# Autodesk Inventor assembly: termoformadora
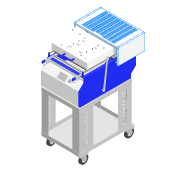
[picture p0: Inventor's stored thumbnail of the model, 180x180]
Saved by Autodesk Inventor 2021 (Build 250183000, 183)
## iProperties
Created: 2021-04-15
Part Number: termoformadora
Document SubType Name: Assembly
Designer: Leonardo Fabio Mercado Benítez
Author: Leonardo Fabio Mercado Benítez
## Documents named in this file (18)
- E:\Documentos\Documentos\Michael_Rodriguez\Universidad_Nacional\Doceaba matricula\PAI\Proyecto PAI\Proyecto_PAI_2021\01 CAD\termoformadora.iam
- E:\Documentos\Documentos\Michael_Rodriguez\Universidad_Nacional\Doceaba matricula\PAI\Proyecto PAI\Proyecto_PAI_2021\01 CAD\Ensamblaje carcasa superior.iam
- E:\Documentos\Documentos\Michael_Rodriguez\Universidad_Nacional\Doceaba matricula\PAI\Proyecto PAI\Proyecto_PAI_2021\01 CAD\soporte_inferior_zona_calor.ipt
- E:\Documentos\Documentos\Michael_Rodriguez\Universidad_Nacional\Doceaba matricula\PAI\Proyecto PAI\Proyecto_PAI_2021\01 CAD\tapa_caja_calor.ipt
- E:\Documentos\Documentos\Michael_Rodriguez\Universidad_Nacional\Doceaba matricula\PAI\Proyecto PAI\Proyecto_PAI_2021\01 CAD\angulo_caja_calor.ipt
- E:\Documentos\Documentos\Michael_Rodriguez\Universidad_Nacional\Doceaba matricula\PAI\Proyecto PAI\Proyecto_PAI_2021\01 CAD\buje_carro_zona_calor.ipt
- E:\Documentos\Documentos\Michael_Rodriguez\Universidad_Nacional\Doceaba matricula\PAI\Proyecto PAI\Proyecto_PAI_2021\01 CAD\barra.ipt
- E:\Documentos\Documentos\Michael_Rodriguez\Universidad_Nacional\Doceaba matricula\PAI\Proyecto PAI\Proyecto_PAI_2021\01 CAD\mango_zona_calor.ipt
- E:\Documentos\Documentos\Michael_Rodriguez\Universidad_Nacional\Doceaba matricula\PAI\Proyecto PAI\Proyecto_PAI_2021\01 CAD\Ensamblaje carcasa control.iam
- E:\Documentos\Documentos\Michael_Rodriguez\Universidad_Nacional\Doceaba matricula\PAI\Proyecto PAI\Proyecto_PAI_2021\01 CAD\soporte_barra.ipt
- E:\Documentos\Documentos\Michael_Rodriguez\Universidad_Nacional\Doceaba matricula\PAI\Proyecto PAI\Proyecto_PAI_2021\01 CAD\ensamble resistencias.iam
- E:\Documentos\Documentos\Michael_Rodriguez\Universidad_Nacional\Doceaba matricula\PAI\Proyecto PAI\Proyecto_PAI_2021\01 CAD\soporte_resistencias.ipt
- E:\Documentos\Documentos\Michael_Rodriguez\Universidad_Nacional\Doceaba matricula\PAI\Proyecto PAI\Proyecto_PAI_2021\01 CAD\Estructura Lámina.iam
- E:\Documentos\Documentos\Michael_Rodriguez\Universidad_Nacional\Doceaba matricula\PAI\Proyecto PAI\Proyecto_PAI_2021\01 CAD\conector_ceramico.ipt
- E:\Documentos\Documentos\Michael_Rodriguez\Universidad_Nacional\Doceaba matricula\PAI\Proyecto PAI\Proyecto_PAI_2021\01 CAD\guarda_conector_ceramico.ipt
- E:\Documentos\Documentos\Michael_Rodriguez\Universidad_Nacional\Doceaba matricula\PAI\Proyecto PAI\Proyecto_PAI_2021\01 CAD\guarda_cables.ipt
- E:\Documentos\Documentos\Michael_Rodriguez\Universidad_Nacional\Doceaba matricula\PAI\Proyecto PAI\Proyecto_PAI_2021\01 CAD\Barras_Soporte_superior.ipt
- C:\Users\Admin\Documents\Inventor\Content Center Files\R2021\es-ES\ISO 7380-1\ISO 7380-1 - M5 x 16.ipt
## Components (34 placed, 17 different names)
1. Ensamblaje carcasa superior:1 [sub-assembly] — Coincidencia:1, Coincidencia:2, Coincidencia:11, Coincidencia:12, Nivelación:7, Coincidencia:16, Coincidencia:17, Coincidencia:57, Coincidencia:58, Coincidencia:59, Coincidencia:60
2. soporte_inferior_zona_calor:1 — Coincidencia:1, Coincidencia:2, Coincidencia:3, Coincidencia:5, Nivelación:3, Nivelación:4, Coincidencia:6, Nivelación:5, Nivelación:6, Coincidencia:15, Insertar:5, Insertar:6, Coincidencia:44, Coincidencia:45, Nivelación:14, Nivelación:15, Ángulo:6, Ángulo:7, Ángulo:8, Ángulo:9, Ángulo:10, Nivelación:16, Coincidencia:56, Nivelación:17
3. tapa_caja_calor:1 — Coincidencia:3, Nivelación:14, Nivelación:15
4. angulo_caja_calor:1 — Coincidencia:5, Nivelación:3, Nivelación:4, Coincidencia:7, Coincidencia:8, Insertar:1, Insertar:2
5. angulo_caja_calor:2 — Coincidencia:6, Nivelación:5, Nivelación:6, Coincidencia:9, Coincidencia:10, Insertar:3, Insertar:4
6. buje_carro_zona_calor:1 — Coincidencia:9, Insertar:3
7. buje_carro_zona_calor:2 — Coincidencia:8, Insertar:2, Coincidencia:14
8. buje_carro_zona_calor:3 — Coincidencia:10, Insertar:4
9. buje_carro_zona_calor:4 — Coincidencia:7, Insertar:1, Coincidencia:13
10. barra:1 — Coincidencia:11, Coincidencia:13, Coincidencia:21
11. barra:2 — Coincidencia:12, Coincidencia:14, Coincidencia:22
12. mango_zona_calor:1 — Coincidencia:15, Insertar:5, Insertar:6
13. Ensamblaje carcasa control:1 [sub-assembly] — Nivelación:7, Coincidencia:16, Coincidencia:17, Nivelación:8, Coincidencia:18, Coincidencia:20, Nivelación:9, Coincidencia:23, Coincidencia:33, Nivelación:10, Nivelación:11
14. soporte_barra:1 — Nivelación:8, Coincidencia:18, Coincidencia:22
15. soporte_barra:2 — Coincidencia:20, Nivelación:9, Coincidencia:21
16. ensamble resistencias:1 [sub-assembly] — Coincidencia:23, Coincidencia:29, Nivelación:12, Nivelación:13
17. soporte_resistencias:1 — Coincidencia:29, Nivelación:12, Nivelación:13, Coincidencia:34, Coincidencia:35, Coincidencia:36, Coincidencia:37, Coincidencia:38, Coincidencia:39, Coincidencia:40, Coincidencia:41, Coincidencia:42, Coincidencia:43, Ángulo:1, Ángulo:2, Ángulo:3, Ángulo:4, Ángulo:5, Coincidencia:44, Coincidencia:45
18. Estructura Lámina:1 [sub-assembly] — Coincidencia:33, Nivelación:10, Nivelación:11
19. conector_ceramico:1 — Coincidencia:37, Coincidencia:42, Ángulo:2, Coincidencia:52
20. conector_ceramico:2 — Coincidencia:36, Coincidencia:41, Ángulo:1, Coincidencia:53
21. conector_ceramico:3 — Coincidencia:34, Coincidencia:39, Ángulo:4, Coincidencia:55
22. conector_ceramico:4 — Coincidencia:38, Coincidencia:43, Ángulo:5, Coincidencia:46, Coincidencia:47, Coincidencia:48, Coincidencia:49, Coincidencia:50, Coincidencia:51
23. conector_ceramico:5 — Coincidencia:35, Coincidencia:40, Ángulo:3, Coincidencia:54
24. guarda_conector_ceramico:1 — Coincidencia:46, Coincidencia:51, Ángulo:10
25. guarda_conector_ceramico:2 — Coincidencia:48, Coincidencia:54, Ángulo:8
26. guarda_conector_ceramico:3 — Coincidencia:47, Coincidencia:52, Ángulo:6
27. guarda_conector_ceramico:4 — Coincidencia:50, Coincidencia:55, Ángulo:9
28. guarda_conector_ceramico:5 — Coincidencia:49, Coincidencia:53, Ángulo:7
29. guarda_cables:1 — Nivelación:16, Coincidencia:56, Nivelación:17
30. Barras_Soporte_superior:1 — Coincidencia:57
31. Barras_Soporte_superior:2 — Coincidencia:58
32. Barras_Soporte_superior:3 — Coincidencia:60
33. Barras_Soporte_superior:4 — Coincidencia:59
34. ISO 7380-1 M5 x 16:4
## Relationships (81: Mate 50, Flush 15, Angle 10, Insert 6)
- Coincidencia:1 [Mate] (61.24 mm): Ensamblaje carcasa superior:1 ↔ soporte_inferior_zona_calor:1
- Coincidencia:2 [Mate] (29 mm): Ensamblaje carcasa superior:1 ↔ soporte_inferior_zona_calor:1
- Coincidencia:3 [Mate]: soporte_inferior_zona_calor:1 ↔ tapa_caja_calor:1
- Coincidencia:5 [Mate]: soporte_inferior_zona_calor:1 ↔ angulo_caja_calor:1
- Nivelación:3 [Flush]: soporte_inferior_zona_calor:1 ↔ angulo_caja_calor:1
- Nivelación:4 [Flush] (10 mm): soporte_inferior_zona_calor:1 ↔ angulo_caja_calor:1
- Coincidencia:6 [Mate]: soporte_inferior_zona_calor:1 ↔ angulo_caja_calor:2
- Nivelación:5 [Flush]: soporte_inferior_zona_calor:1 ↔ angulo_caja_calor:2
- Nivelación:6 [Flush]: soporte_inferior_zona_calor:1 ↔ angulo_caja_calor:2
- Coincidencia:7 [Mate]: angulo_caja_calor:1 ↔ buje_carro_zona_calor:4
- Coincidencia:8 [Mate]: angulo_caja_calor:1 ↔ buje_carro_zona_calor:2
- Coincidencia:9 [Mate]: angulo_caja_calor:2 ↔ buje_carro_zona_calor:1
- Coincidencia:10 [Mate]: angulo_caja_calor:2 ↔ buje_carro_zona_calor:3
- Insertar:1: angulo_caja_calor:1 ↔ buje_carro_zona_calor:4
- Insertar:2: angulo_caja_calor:1 ↔ buje_carro_zona_calor:2
- Insertar:3: angulo_caja_calor:2 ↔ buje_carro_zona_calor:1
- Insertar:4: angulo_caja_calor:2 ↔ buje_carro_zona_calor:3
- Coincidencia:11 [Mate]: Ensamblaje carcasa superior:1 ↔ barra:1
- Coincidencia:12 [Mate]: Ensamblaje carcasa superior:1 ↔ barra:2
- Coincidencia:13 [Mate]: buje_carro_zona_calor:4 ↔ barra:1
- Coincidencia:14 [Mate]: buje_carro_zona_calor:2 ↔ barra:2
- Coincidencia:15 [Mate]: soporte_inferior_zona_calor:1 ↔ mango_zona_calor:1
- Insertar:5: soporte_inferior_zona_calor:1 ↔ mango_zona_calor:1
- Insertar:6: soporte_inferior_zona_calor:1 ↔ mango_zona_calor:1
- Nivelación:7 [Flush] (-74.1 mm): Ensamblaje carcasa superior:1 ↔ Ensamblaje carcasa control:1
- Coincidencia:16 [Mate] (-43.5 mm): Ensamblaje carcasa superior:1 ↔ Ensamblaje carcasa control:1
- Coincidencia:17 [Mate] (53.74 mm): Ensamblaje carcasa superior:1 ↔ Ensamblaje carcasa control:1
- Nivelación:8 [Flush] (5 mm): Ensamblaje carcasa control:1 ↔ soporte_barra:1
- Coincidencia:18 [Mate]: Ensamblaje carcasa control:1 ↔ soporte_barra:1
- Coincidencia:20 [Mate]: Ensamblaje carcasa control:1 ↔ soporte_barra:2
- Nivelación:9 [Flush] (5 mm): Ensamblaje carcasa control:1 ↔ soporte_barra:2
- Coincidencia:21 [Mate]: barra:1 ↔ soporte_barra:2
- Coincidencia:22 [Mate]: barra:2 ↔ soporte_barra:1
- Coincidencia:23 [Mate] (106 mm): Ensamblaje carcasa control:1 ↔ ensamble resistencias:1
- Coincidencia:29 [Mate]: ensamble resistencias:1 ↔ soporte_resistencias:1
- Coincidencia:33 [Mate]: Ensamblaje carcasa control:1 ↔ Estructura Lámina:1
- Nivelación:10 [Flush] (10 mm): Ensamblaje carcasa control:1 ↔ Estructura Lámina:1
- Nivelación:11 [Flush]: Ensamblaje carcasa control:1 ↔ Estructura Lámina:1
- Nivelación:12 [Flush] (33.5 mm): ensamble resistencias:1 ↔ soporte_resistencias:1
- Nivelación:13 [Flush] (34 mm): ensamble resistencias:1 ↔ soporte_resistencias:1
- Coincidencia:34 [Mate]: soporte_resistencias:1 ↔ conector_ceramico:3
- Coincidencia:35 [Mate]: soporte_resistencias:1 ↔ conector_ceramico:5
- Coincidencia:36 [Mate]: soporte_resistencias:1 ↔ conector_ceramico:2
- Coincidencia:37 [Mate]: soporte_resistencias:1 ↔ conector_ceramico:1
- Coincidencia:38 [Mate]: soporte_resistencias:1 ↔ conector_ceramico:4
- Coincidencia:39 [Mate]: soporte_resistencias:1 ↔ conector_ceramico:3
- Coincidencia:40 [Mate]: soporte_resistencias:1 ↔ conector_ceramico:5
- Coincidencia:41 [Mate]: soporte_resistencias:1 ↔ conector_ceramico:2
- Coincidencia:42 [Mate]: soporte_resistencias:1 ↔ conector_ceramico:1
- Coincidencia:43 [Mate]: soporte_resistencias:1 ↔ conector_ceramico:4
- Ángulo:1 [Angle] (0 deg): soporte_resistencias:1 ↔ conector_ceramico:2
- Ángulo:2 [Angle] (0 deg): soporte_resistencias:1 ↔ conector_ceramico:1
- Ángulo:3 [Angle] (0 deg): soporte_resistencias:1 ↔ conector_ceramico:5
- Ángulo:4 [Angle] (0 deg): soporte_resistencias:1 ↔ conector_ceramico:3
- Ángulo:5 [Angle] (0 deg): soporte_resistencias:1 ↔ conector_ceramico:4
- Coincidencia:44 [Mate] (0.5 mm): soporte_inferior_zona_calor:1 ↔ soporte_resistencias:1
- Coincidencia:45 [Mate] (0.5 mm): soporte_inferior_zona_calor:1 ↔ soporte_resistencias:1
- Nivelación:14 [Flush] (25.4 mm): soporte_inferior_zona_calor:1 ↔ tapa_caja_calor:1
- Nivelación:15 [Flush] (31.75 mm): soporte_inferior_zona_calor:1 ↔ tapa_caja_calor:1
- Coincidencia:46 [Mate]: conector_ceramico:4 ↔ guarda_conector_ceramico:1
- Coincidencia:47 [Mate]: conector_ceramico:4 ↔ guarda_conector_ceramico:3
- Coincidencia:48 [Mate]: conector_ceramico:4 ↔ guarda_conector_ceramico:2
- Coincidencia:49 [Mate]: conector_ceramico:4 ↔ guarda_conector_ceramico:5
- Coincidencia:50 [Mate]: conector_ceramico:4 ↔ guarda_conector_ceramico:4
- Coincidencia:51 [Mate]: conector_ceramico:4 ↔ guarda_conector_ceramico:1
- Coincidencia:52 [Mate]: conector_ceramico:1 ↔ guarda_conector_ceramico:3
- Coincidencia:53 [Mate]: conector_ceramico:2 ↔ guarda_conector_ceramico:5
- Coincidencia:54 [Mate]: conector_ceramico:5 ↔ guarda_conector_ceramico:2
- Coincidencia:55 [Mate]: conector_ceramico:3 ↔ guarda_conector_ceramico:4
- Ángulo:6 [Angle] (0 deg): soporte_inferior_zona_calor:1 ↔ guarda_conector_ceramico:3
- Ángulo:7 [Angle] (0 deg): soporte_inferior_zona_calor:1 ↔ guarda_conector_ceramico:5
- Ángulo:8 [Angle] (0 deg): soporte_inferior_zona_calor:1 ↔ guarda_conector_ceramico:2
- Ángulo:9 [Angle] (0 deg): soporte_inferior_zona_calor:1 ↔ guarda_conector_ceramico:4
- Ángulo:10 [Angle] (0 deg): soporte_inferior_zona_calor:1 ↔ guarda_conector_ceramico:1
- Nivelación:16 [Flush]: soporte_inferior_zona_calor:1 ↔ guarda_cables:1
- Coincidencia:56 [Mate]: soporte_inferior_zona_calor:1 ↔ guarda_cables:1
- Nivelación:17 [Flush]: soporte_inferior_zona_calor:1 ↔ guarda_cables:1
- Coincidencia:57 [Mate]: Ensamblaje carcasa superior:1 ↔ Barras_Soporte_superior:1
- Coincidencia:58 [Mate]: Ensamblaje carcasa superior:1 ↔ Barras_Soporte_superior:2
- Coincidencia:59 [Mate]: Ensamblaje carcasa superior:1 ↔ Barras_Soporte_superior:4
- Coincidencia:60 [Mate]: Ensamblaje carcasa superior:1 ↔ Barras_Soporte_superior:3
